# Autodesk Inventor assembly: Povorot_mec.ipt
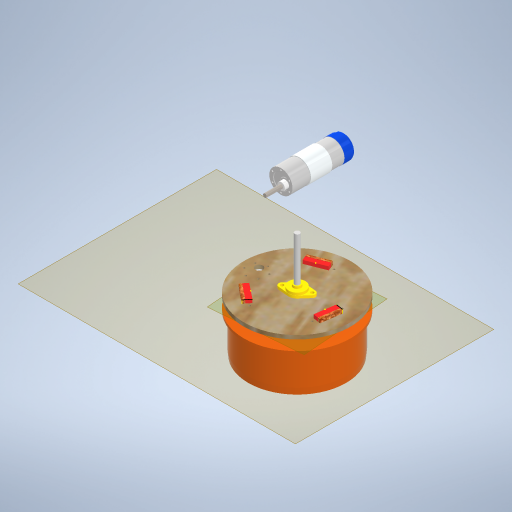
[picture p0: Inventor's stored thumbnail of the model, 512x512]
Saved by Autodesk Inventor 2023 (Build 270158000, 158)
## iProperties
Created: 2023-12-24
Part Number: Povorot_mec.ipt
Document SubType Name: Assembly
Designer: Dell
Author: Dell
## Documents named in this file (16)
- C:\Fox_Crow\Work\Crow_Sborka\Поворотный механизм\Поворотный Механизм.iam
- C:\Fox_Crow\Work\Crow_Sborka\Поворотный механизм\Pitsco Education-739085.ipt
- C:\Fox_Crow\Work\Crow_Sborka\Поворотный механизм\Cap_pipes.ipt
- C:\Fox_Crow\Work\Crow_Sborka\Поворотный механизм\Pitsco Education-739028.ipt
- C:\Fox_Crow\Work\Crow_Sborka\Поворотный механизм\Fanerka.ipt
- C:\Fox_Crow\Work\Crow_Sborka\Поворотный механизм\Prostavka.ipt
- C:\Fox_Crow\Work\Crow_Sborka\Поворотный механизм\Det_podsh.ipt
- C:\Fox_Crow\Work\Crow_Sborka\Поворотный механизм\Podsh.ipt
- C:\Fox_Crow\Work\Crow_Sborka\Поворотный механизм\User Library-Bearing KFL08.ipt
- C:\Fox_Crow\Work\Crow_Sborka\Поворотный механизм\trubka.ipt
- C:\Users\Dell\Downloads\User Library-DC gearhead motor.ipt
- C:\Fox_Crow\Work\Crow_Sborka\Поворотный механизм\39079_TXM-Motor Shaft Hub With Set Screw.ipt
- C:\Fox_Crow\Work\Crow_Sborka\Поворотный механизм\SHF8 Горизонтальный держатель вала.ipt
- C:\Fox_Crow\Work\Crow_Sborka\Поворотный механизм\ISO 14583 — M5x16-4.8.ipt
- C:\Fox_Crow\Work\Crow_Sborka\Поворотный механизм\ISO 7046-1 - M6 x 20_ - 4.8 - H - ISO.ipt
- C:\Fox_Crow\Work\Crow_Sborka\Поворотный механизм\44260_txm torquenado dc motor.ipt
## Components (23 placed, 15 different names)
1. Pitsco Education-739085:1 — Жесткий:6, Совмещение:10, Совмещение:11, Совмещение:13, Совмещение:16
2. Cap_pipes:1 — Цилиндрический:2, Совмещение:8, Совмещение:9
3. Pitsco Education-739028:1
4. Fanerka:1 — Совмещение:9, Плоский:1, Плоский:2, Плоский:3, Цилиндрический:4, С поворотом:3, С поворотом:4, Совмещение:17
5. Prostavka:1 — Цилиндрический:2, Совмещение:8, Жесткий:5
6. User Library-Bearing KFL08:1 — С поворотом:3, С поворотом:4
7. trubka:1 — Жесткий:5, Жесткий:6, Цилиндрический:5
8. User Library-DC gearhead motor:1 — Цилиндрический:4, Жесткий:7
9. 39079_TXM-Motor Shaft Hub With Set Screw:1 — Жесткий:7
10. Винт ISO 14583:2011(E) M5x16-4.8:2
11. Винт ISO 14583:2011(E) M5x16-4.8:3
12. SHF8 Горизонтальный держатель вала:3 — Цилиндрический:5
13. ISO 7046-1 H M6 x 20 - 4.8 - H:1 — Совмещение:10
14. ISO 7046-1 H M6 x 20 - 4.8 - H:2 — Совмещение:11
15. ISO 7046-1 H M6 x 20 - 4.8 - H:3 — Совмещение:13
16. ISO 7046-1 H M6 x 20 - 4.8 - H:4 — Совмещение:16
17. 44260_txm torquenado dc motor:1 — Совмещение:17
18. Det_podsh:2 — С поворотом:1, Плоский:1, Плоский:2, Плоский:3
19. Podsh:1 — С поворотом:1
20. Det_podsh:3
21. Podsh:2
22. Det_podsh:4
23. Podsh:3
## Component patterns: (3 elements, first: Det_podsh:2 + Podsh:1)
## Relationships (19: Mate 7, CylindricalJoint 3, RevoluteJoint 3, PlanarJoint 3, WeldJoint 3)
- Цилиндрический:2 [CylindricalJoint]: Cap_pipes:1 ↔ Prostavka:1
- Совмещение:8 [Mate]: Cap_pipes:1 ↔ Prostavka:1
- Совмещение:9 [Mate]: Cap_pipes:1 ↔ Fanerka:1
- С поворотом:1 [RevoluteJoint]: Det_podsh:2 ↔ Podsh:1
- Плоский:1 [PlanarJoint]: Fanerka:1 ↔ Det_podsh:2
- Плоский:2 [PlanarJoint]: Fanerka:1 ↔ Det_podsh:2
- Плоский:3 [PlanarJoint]: Fanerka:1 ↔ Det_podsh:2
- Жесткий:5 [WeldJoint]: Prostavka:1 ↔ trubka:1
- Жесткий:6 [WeldJoint]: Pitsco Education-739085:1 ↔ trubka:1
- Цилиндрический:4 [CylindricalJoint]: Fanerka:1 ↔ User Library-DC gearhead motor:1
- Жесткий:7 [WeldJoint]: User Library-DC gearhead motor:1 ↔ 39079_TXM-Motor Shaft Hub With Set Screw:1
- С поворотом:3 [RevoluteJoint]: Fanerka:1 ↔ User Library-Bearing KFL08:1
- С поворотом:4 [RevoluteJoint]: Fanerka:1 ↔ User Library-Bearing KFL08:1
- Цилиндрический:5 [CylindricalJoint]: trubka:1 ↔ SHF8 Горизонтальный держатель вала:3
- Совмещение:10 [Mate]: Pitsco Education-739085:1 ↔ ISO 7046-1 H M6 x 20 - 4.8 - H:1
- Совмещение:11 [Mate]: Pitsco Education-739085:1 ↔ ISO 7046-1 H M6 x 20 - 4.8 - H:2
- Совмещение:13 [Mate]: Pitsco Education-739085:1 ↔ ISO 7046-1 H M6 x 20 - 4.8 - H:3
- Совмещение:16 [Mate]: Pitsco Education-739085:1 ↔ ISO 7046-1 H M6 x 20 - 4.8 - H:4
- Совмещение:17 [Mate]: Fanerka:1 ↔ 44260_txm torquenado dc motor:1
